# Autodesk Inventor assembly: BOX_PART
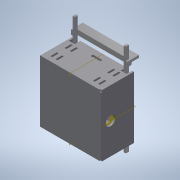
[picture p0: Inventor's stored thumbnail of the model, 180x180]
Saved by Autodesk Inventor 2020 (Build 240168000, 168)
## iProperties
Created: 2019-12-17
Part Number: BOX_PART
Document SubType Name: Assembly
Designer: fabfarm
Author: fabfarm
## Documents named in this file (6)
- D:\fablab\save\Scisor\BOX_PART.iam
- D:\fablab\save\Scisor\Side_one.ipt
- D:\fablab\save\Scisor\Side_two.ipt
- D:\fablab\save\Scisor\TableSaw_Bench3.ipt
- D:\fablab\save\Scisor\bottom-case.ipt
- D:\fablab\save\Scisor\open_case.ipt
## Components (6 placed, 5 different names)
1. Side_one:1 — Mate:12, Flush:4, Flush:5, Symmetry:1, Placage:16, Placage:17
2. Side_two:1 — Mate:10, Mate:12, Flush:4, Flush:7, Symmetry:2, Placage:16, Placage:18
3. TableSaw_Bench3:1 — Flush:6, Flush:9, Affleurement:11
4. Side_one:2 — Flush:6, Flush:7, Flush:8, Flush:10, Symmetry:1, Placage:13, Placage:14, Placage:19
5. bottom-case:1 — Mate:10, Flush:5, Flush:8, Placage:14, Placage:17
6. open_case:1 — Flush:9, Flush:10, Symmetry:2, Placage:13
## Relationships (18: Mate 8, Flush 8, Symmetry 2)
- Mate:10: Side_two:1 ↔ bottom-case:1
- Mate:12: Side_one:1 ↔ Side_two:1
- Flush:4: Side_one:1 ↔ Side_two:1
- Flush:5: Side_one:1 ↔ bottom-case:1
- Flush:6: TableSaw_Bench3:1 ↔ Side_one:2
- Flush:7: Side_two:1 ↔ Side_one:2
- Flush:8: Side_one:2 ↔ bottom-case:1
- Flush:9: TableSaw_Bench3:1 ↔ open_case:1
- Flush:10: Side_one:2 ↔ open_case:1
- Symmetry:1: Side_one:1 ↔ Side_one:2
- Symmetry:2: Side_two:1 ↔ open_case:1
- Placage:13 [Mate]: Side_one:2 ↔ open_case:1
- Placage:14 [Mate]: Side_one:2 ↔ bottom-case:1
- Placage:16 [Mate]: Side_one:1 ↔ Side_two:1
- Placage:17 [Mate]: Side_one:1 ↔ bottom-case:1
- Affleurement:11 [Flush]: TableSaw_Bench3:1
- Placage:18 [Mate]: Side_two:1
- Placage:19 [Mate]: Side_one:2
